# Autodesk Inventor assembly: Jose_Ensamble_Set_Sobre_Robot
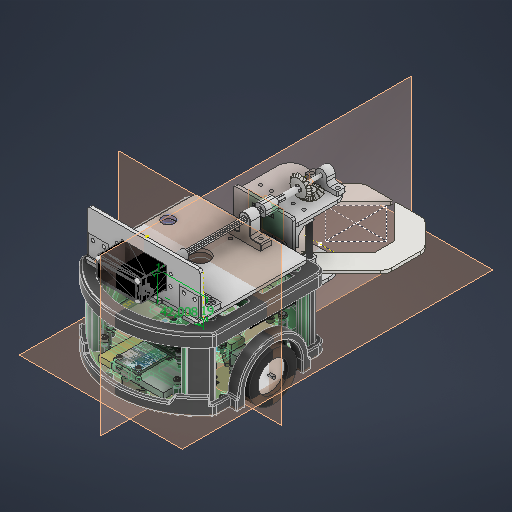
[picture p0: Inventor's stored thumbnail of the model, 512x512]
Saved by Autodesk Inventor 2026.3 (Build 303398000, 398)
## iProperties
Created: 2025-10-21
Part Number: Jose_Ensamble_Set_Sobre_Robot
Document SubType Name: Assembly
Designer: brene
Author: brene
## Documents named in this file (50)
- C:\Users\Caro\JoseCarlos\TEC\TFG\Inventor\PiezasSTD\Jose_Ensamble_Set_Sobre_Robot.iam
- C:\Users\Caro\JoseCarlos\TEC\TFG\Inventor\AttaBotStemV3\Diseño V3.0\base_chasis_v6\base_chasis_v4-dimsAjustadas.ipt
- C:\Users\Caro\JoseCarlos\TEC\TFG\Inventor\AttaBotStemV3\Diseño V3.0\base_chasis_v6.ipt
- C:\Users\Caro\JoseCarlos\TEC\TFG\Inventor\AttaBotStemV3\Diseño V3.0\Content Center Files\en-US\ISO 4762(2)\ISO 4762 - M2 x 12ISO.ipt
- C:\Users\Caro\JoseCarlos\TEC\TFG\Inventor\AttaBotStemV3\Diseño V3.0\switch.ipt
- C:\Users\Caro\JoseCarlos\TEC\TFG\Inventor\AttaBotStemV3\Diseño V3.0\Content Center Files\en-US\ISO 4762(2)\ISO 4762 - M2 x 8ISO.ipt
- C:\Users\Caro\JoseCarlos\TEC\TFG\Inventor\AttaBotStemV3\Diseño V3.0\Content Center Files\en-US\ISO 4032(2)\ISO 4032 - M2 - ISO.ipt
- C:\Users\Caro\JoseCarlos\TEC\TFG\Inventor\AttaBotStemV3\Diseño V3.0\ball_caster.ipt
- C:\Users\Caro\JoseCarlos\TEC\TFG\Inventor\AttaBotStemV3\Diseño V3.0\sensorInferior.ipt
- C:\Users\Caro\JoseCarlos\TEC\TFG\Inventor\AttaBotStemV3\Diseño V3.0\Content Center Files\en-US\ISO 4762(2)\ISO 4762 - M3 x 12ISO.ipt
- C:\Users\Caro\JoseCarlos\TEC\TFG\Inventor\AttaBotStemV3\Diseño V3.0\Content Center Files\en-US\ISO 4032(2)\ISO 4032 - M3 - ISO.ipt
- C:\Users\Caro\JoseCarlos\TEC\TFG\Inventor\AttaBotStemV3\Diseño V3.0\spacers\hexagonal_spacer_MF_M3_H20_HEX5.5_FTD6_MTL6.ipt
- C:\Users\Caro\JoseCarlos\TEC\TFG\Inventor\AttaBotStemV3\Diseño V3.0\spacers\hexagonal_spacer_MF_M3_H06_HEX5.5_FTD3_MTL6.ipt
- C:\Users\Caro\JoseCarlos\TEC\TFG\Inventor\AttaBotStemV3\Diseño V3.0\Content Center Files\en-US\ISO 4762(2)\ISO 4762 - M3 x 8ISO.ipt
- C:\Users\Caro\JoseCarlos\TEC\TFG\Inventor\AttaBotStemV3\Diseño V3.0\spacers\hexagonal_spacer_MF_M3_H08_HEX5_FTD4_MTL8.ipt
- C:\Users\Caro\JoseCarlos\TEC\TFG\Inventor\AttaBotStemV3\Diseño V3.0\bateria.ipt
- C:\Users\Caro\JoseCarlos\TEC\TFG\Inventor\AttaBotStemV3\Diseño V3.0\base_powerboost.ipt
- C:\Users\Caro\JoseCarlos\TEC\TFG\Inventor\AttaBotStemV3\Diseño V3.0\powerboost.ipt
- C:\Users\Caro\JoseCarlos\TEC\TFG\Inventor\AttaBotStemV3\Diseño V3.0\base_nivel2.ipt
- C:\Users\Caro\JoseCarlos\TEC\TFG\Inventor\AttaBotStemV3\Diseño V3.0\ideaboard.ipt
- C:\Users\Caro\JoseCarlos\TEC\TFG\Inventor\AttaBotStemV3\Diseño V3.0\sensorFrontal.ipt
- C:\Users\Caro\JoseCarlos\TEC\TFG\Inventor\AttaBotStemV3\Diseño V3.0\Tower Pro MG90S Micro servo.ipt
- C:\Users\Caro\JoseCarlos\TEC\TFG\Inventor\AttaBotStemV3\Diseño V3.0\spacers\hexagonal_spacer_MF_M3_H10_HEX5.5_FTD6_MTL6.ipt
- C:\Users\Caro\JoseCarlos\TEC\TFG\Inventor\AttaBotStemV3\Diseño V3.0\SoporteMotor_3.0.ipt
- C:\Users\Caro\JoseCarlos\TEC\TFG\Inventor\AttaBotStemV3\Diseño V3.0\motor.ipt
- C:\Users\Caro\JoseCarlos\TEC\TFG\Inventor\AttaBotStemV3\Diseño V3.0\llanta.ipt
- C:\Users\Caro\JoseCarlos\TEC\TFG\Inventor\AttaBotStemV3\Diseño V3.0\Unidirectional shoulder.ipt
- C:\Users\Caro\JoseCarlos\TEC\TFG\Inventor\AttaBotStemV3\Diseño V3.0\SujecionServo.ipt
- C:\Users\06aar\Documents\Inventor\Content Center Files\R2026\en-US\SS-ISO 4762\ISO 4762 - M2,5 x 25SS-ISO.ipt
- C:\Users\Caro\JoseCarlos\TEC\TFG\Inventor\AttaBotStemV3\Diseño V3.0\Esquinero Trasero\base_chasis_v4-dimsAjustadas.ipt
- C:\Users\Caro\JoseCarlos\TEC\TFG\Inventor\AttaBotStemV3\Diseño V3.0\Esquinero Trasero.ipt
- C:\Users\Caro\JoseCarlos\TEC\TFG\Inventor\AttaBotStemV3\Diseño V3.0\Bumper Trasero\base_chasis_v4-dimsAjustadas.ipt
- C:\Users\Caro\JoseCarlos\TEC\TFG\Inventor\AttaBotStemV3\Diseño V3.0\Bumper Trasero.ipt
- C:\Users\Caro\JoseCarlos\TEC\TFG\Inventor\AttaBotStemV3\Diseño V3.0\Guardabarros.ipt
- C:\Users\Caro\JoseCarlos\TEC\TFG\Inventor\AttaBotStemV3\Diseño V3.0\Bumper Delantero.ipt
- C:\Users\Caro\JoseCarlos\TEC\TFG\Inventor\AttaBotStemV3\Diseño V3.0\Esquineros Delanteros.ipt
- C:\Users\Caro\JoseCarlos\TEC\TFG\Inventor\AttaBotStemV3\Diseño V3.0\PARED TRASERA.ipt
- C:\Users\Caro\JoseCarlos\TEC\TFG\Inventor\AttaBotStemV3\Diseño V3.0\PAREDES LATERALES.ipt
- C:\Users\Caro\JoseCarlos\TEC\TFG\Inventor\AttaBotStemV3\Diseño V3.0\PAREDES LATERALES_MIR.ipt
- C:\Users\Caro\JoseCarlos\TEC\TFG\Inventor\AttaBotStemV3\Diseño V3.0\PARED FRONTAL.ipt
- C:\Users\Caro\JoseCarlos\TEC\TFG\Inventor\AttaBotStemV3\Diseño V3.0\Techo Armadura.ipt
- C:\Users\Caro\JoseCarlos\TEC\TFG\Inventor\AttaBotStemV3\Diseño V3.0\Acrilicos Superiores.ipt
- C:\Users\Caro\JoseCarlos\TEC\TFG\Inventor\AttaBotStemV3\Diseño V3.0\Pieza de Silicona.ipt
- C:\Users\Caro\JoseCarlos\TEC\TFG\Inventor\AttaBotStemV3\Diseño V3.0\PresaPilotInventorVersion.ipt
- C:\Users\Caro\JoseCarlos\TEC\TFG\Inventor\AttaBotStemV3\Diseño V3.0\spacers\hexagonal_spacer_MF_M3_H20_HEX5.5_FTD6_MTL6_MIR.ipt
- C:\Users\Caro\JoseCarlos\TEC\TFG\Inventor\PiezasSTD\BaseMotorSetJose.ipt
- C:\Users\Caro\JoseCarlos\TEC\TFG\Inventor\PiezasSTD\EnsambleGarraSTD.iam
- C:\Users\Caro\JoseCarlos\TEC\TFG\Inventor\PiezasSTD\DistanciaSpacer3mm.ipt
- C:\Users\Caro\JoseCarlos\TEC\TFG\Inventor\PiezasSTD\EnsambleMotor\EnsambleBaseMotor.iam
- C:\Users\Caro\JoseCarlos\TEC\TFG\Inventor\PiezasSTD\EnsambleMotor\EjeMotor.ipt
## Components (120 placed, 44 different names)
1. BaseMotorSetJose:1 — Nivelación:215
2. EnsambleGarraSTD:1 [sub-assembly] — Coincidencia:293, Nivelación:220, Coincidencia:294, Nivelación:222
3. DistanciaSpacer3mm:1 — Nivelación:219, Coincidencia:293
4. EjeMotor:1 — Nivelación:222
5. EnsambleBaseMotor_Mediciones [sub-assembly] — Ángulo:7, Coincidencia:299, Coincidencia:300, Ángulo:8
6. hexagonal_spacer_MF_M3_H20_HEX5.5_FTD6_MTL6:5 — Coincidencia:289, Coincidencia:290
7. hexagonal_spacer_MF_M3_H20_HEX5.5_FTD6_MTL6_MIR:1
8. ISO 4762 M3 x 8:10 — Coincidencia:151, Coincidencia:152
9. ISO 4762 M3 x 8:9 — Coincidencia:153, Coincidencia:154, Coincidencia:285
10. hexagonal_spacer_MF_M3_H10_HEX5.5_FTD6_MTL6:2 — Coincidencia:148, Coincidencia:150
11. hexagonal_spacer_MF_M3_H10_HEX5.5_FTD6_MTL6:1 — Coincidencia:147, Coincidencia:149
12. ISO 4762 M3 x 8:8 — Coincidencia:113, Coincidencia:114, Coincidencia:250, Coincidencia:251
13. ISO 4762 M3 x 8:7 — Coincidencia:117, Coincidencia:118
14. ISO 4032 M3:8 — Coincidencia:123, Coincidencia:124
15. ISO 4032 M3:7 — Coincidencia:125, Coincidencia:126
16. hexagonal_spacer_MF_M3_H06_HEX5.5_FTD3_MTL6:10 — Coincidencia:115, Coincidencia:116, Coincidencia:119, Coincidencia:120, Coincidencia:126
17. hexagonal_spacer_MF_M3_H06_HEX5.5_FTD3_MTL6:9 — Coincidencia:111, Coincidencia:112, Coincidencia:121, Coincidencia:122, Coincidencia:124
18. hexagonal_spacer_MF_M3_H06_HEX5.5_FTD3_MTL6:8 — Coincidencia:104, Coincidencia:105, Coincidencia:108, Coincidencia:110, Coincidencia:132, Coincidencia:175
19. hexagonal_spacer_MF_M3_H06_HEX5.5_FTD3_MTL6:7 — Coincidencia:106, Coincidencia:107, Coincidencia:134, Coincidencia:177
20. hexagonal_spacer_MF_M3_H06_HEX5.5_FTD3_MTL6:6 — Coincidencia:100, Coincidencia:101, Coincidencia:109, Coincidencia:130, Coincidencia:179, Coincidencia:275, Coincidencia:276, Coincidencia:277, Coincidencia:278, Coincidencia:279, Coincidencia:280, Coincidencia:281
21. hexagonal_spacer_MF_M3_H06_HEX5.5_FTD3_MTL6:5 — Coincidencia:102, Coincidencia:103, Coincidencia:128, Coincidencia:181
22. ISO 4762 M3 x 8:6 — Coincidencia:94, Coincidencia:95
23. ISO 4762 M3 x 8:5 — Coincidencia:96, Coincidencia:97
24. ISO 4762 M3 x 8:4 — Coincidencia:92, Coincidencia:93
25. ISO 4762 M3 x 8:3 — Coincidencia:98, Coincidencia:99
26. ISO 4032 M2:10 — Coincidencia:84, Coincidencia:85
27. ISO 4032 M2:9 — Coincidencia:80, Coincidencia:81
28. ISO 4032 M2:8 — Coincidencia:86, Coincidencia:87
29. ISO 4032 M2:7 — Coincidencia:82, Coincidencia:83
30. ISO 4032 M2:6 — Coincidencia:64, Coincidencia:65, Coincidencia:70
31. ISO 4032 M2:5 — Coincidencia:66, Coincidencia:67
32. ISO 4032 M2:4 — Coincidencia:62, Coincidencia:63, Coincidencia:71
33. ISO 4032 M2:3 — Coincidencia:68, Coincidencia:69
34. ISO 4762 M2 x 8:6 — Coincidencia:76, Coincidencia:77, Coincidencia:87, Coincidencia:91
35. ISO 4762 M2 x 8:5 — Coincidencia:78, Coincidencia:79, Coincidencia:85
36. ISO 4762 M2 x 12:2 — Coincidencia:72, Coincidencia:73, Coincidencia:83
37. ISO 4762 M2 x 12:1 — Coincidencia:74, Coincidencia:75, Coincidencia:81
38. ISO 4032 M3:6 — Coincidencia:48, Coincidencia:49, Coincidencia:57
39. ISO 4032 M3:5 — Coincidencia:50, Coincidencia:51, Coincidencia:59
40. ISO 4032 M3:4 — Coincidencia:46, Coincidencia:47, Coincidencia:53
41. ISO 4032 M3:3 — Coincidencia:44, Coincidencia:45, Coincidencia:55
42. hexagonal_spacer_MF_M3_H08_HEX5_FTD4_MTL8:4 — Coincidencia:54, Coincidencia:55, Coincidencia:90
43. hexagonal_spacer_MF_M3_H08_HEX5_FTD4_MTL8:3 — Coincidencia:52, Coincidencia:53, Coincidencia:89
44. hexagonal_spacer_MF_M3_H08_HEX5_FTD4_MTL8:2 — Coincidencia:58, Coincidencia:59, Coincidencia:88
45. hexagonal_spacer_MF_M3_H08_HEX5_FTD4_MTL8:1 — Coincidencia:56, Coincidencia:57, Coincidencia:61
46. ISO 4762 M3 x 8:2 — Coincidencia:34, Coincidencia:35, Coincidencia:39
47. ISO 4762 M3 x 8:1 — Coincidencia:32, Coincidencia:33, Coincidencia:37
48. hexagonal_spacer_MF_M3_H20_HEX5.5_FTD6_MTL6:4 — Coincidencia:36, Coincidencia:37, Coincidencia:137, Coincidencia:145
49. hexagonal_spacer_MF_M3_H20_HEX5.5_FTD6_MTL6:3 — Coincidencia:38, Coincidencia:39, Coincidencia:143
50. hexagonal_spacer_MF_M3_H20_HEX5.5_FTD6_MTL6:2 — Coincidencia:26, Coincidencia:27, Coincidencia:135, Coincidencia:141
51. hexagonal_spacer_MF_M3_H20_HEX5.5_FTD6_MTL6:1 — Coincidencia:24, Coincidencia:25, Coincidencia:136, Coincidencia:139
52. ISO 4032 M3:2 — Coincidencia:14, Coincidencia:15, Coincidencia:23
53. ISO 4032 M3:1 — Coincidencia:12, Coincidencia:13, Coincidencia:21
54. ISO 4762 M3 x 12:2 — Coincidencia:23, Coincidencia:27
55. ISO 4762 M3 x 12:1 — Coincidencia:21, Coincidencia:25, Coincidencia:283
56. ISO 4762 M2 x 8:4 — Coincidencia:8, Coincidencia:9, Tangente:4
57. ISO 4762 M2 x 8:3 — Coincidencia:10, Coincidencia:11, Tangente:3
58. ISO 4032 M2:2 — Insertar:2
59. ISO 4032 M2:1 — Insertar:1
60. ISO 4762 M2 x 8:2 — Coincidencia:3, Coincidencia:4
61. ISO 4762 M2 x 8:1 — Coincidencia:5, Coincidencia:6
62. ISO 4032 M3:16 — Coincidencia:144, Coincidencia:145
63. ISO 4032 M3:15 — Coincidencia:140, Coincidencia:141
64. ISO 4032 M3:14 — Coincidencia:138, Coincidencia:139
65. ISO 4032 M3:13 — Coincidencia:142, Coincidencia:143
66. ISO 4032 M3:12 — Coincidencia:127, Coincidencia:128
67. ISO 4032 M3:11 — Coincidencia:131, Coincidencia:132
68. ISO 4032 M3:10 — Coincidencia:129, Coincidencia:130
69. ISO 4032 M3:9 — Coincidencia:133, Coincidencia:134
70. ISO 4032 M2:15 — Coincidencia:194, Coincidencia:195
71. ISO 4032 M2:14 — Coincidencia:196, Coincidencia:197
72. ISO 4032 M2:13 — Coincidencia:192, Coincidencia:193
73. ISO 4032 M2:12 — Coincidencia:190, Coincidencia:191
74. ISO 4762 M2 x 8:10 — Coincidencia:183, Coincidencia:197
75. ISO 4762 M2 x 8:9 — Coincidencia:187, Coincidencia:193
76. ISO 4762 M2 x 8:8 — Coincidencia:189, Coincidencia:191
77. ISO 4762 M2 x 8:7 — Coincidencia:185, Coincidencia:195
78. ISO 4762 M3 x 8:14 — Coincidencia:174, Coincidencia:175
79. ISO 4762 M3 x 8:13 — Coincidencia:178, Coincidencia:179
80. ISO 4762 M3 x 8:12 — Coincidencia:180, Coincidencia:181, Coincidencia:274
81. ISO 4762 M3 x 8:11 — Coincidencia:176, Coincidencia:177
82. SS ISO 4762 M2,5 x 25:12 — Insert:18, Coincidencia:282
83. SS ISO 4762 M2,5 x 25:11 — Insert:17
84. SS ISO 4762 M2,5 x 25:9 — Insert:15
85. SS ISO 4762 M2,5 x 25:8 — Insert:14
86. SS ISO 4762 M2,5 x 25:6 — Insert:12
87. SS ISO 4762 M2,5 x 25:4 — Insert:10
88. sensorInferior:3 — Coincidencia:282, Coincidencia:283, Coincidencia:284
89. switch:1 — Coincidencia:1, Coincidencia:2, Coincidencia:3, Coincidencia:5, Ángulo:3
90. ball_caster:1 — Coincidencia:7, Tangente:1, Tangente:2, Coincidencia:9, Coincidencia:11
91. bateria:1 — Coincidencia:60, Coincidencia:61, Coincidencia:146, Ángulo:2
92. base_powerboost:1 — Coincidencia:62, Coincidencia:63, Coincidencia:64, Coincidencia:65, Coincidencia:66, Coincidencia:67, Coincidencia:68, Coincidencia:69, Coincidencia:80, Coincidencia:82, Coincidencia:84, Coincidencia:86, Coincidencia:88, Coincidencia:89, Coincidencia:90, Coincidencia:91, Coincidencia:92, Coincidencia:93, Coincidencia:94, Coincidencia:95, Coincidencia:96, Coincidencia:97, Coincidencia:98, Coincidencia:99
93. powerboost:1 — Coincidencia:70, Coincidencia:71, Coincidencia:72, Coincidencia:73, Coincidencia:74, Coincidencia:75, Coincidencia:76, Coincidencia:77, Coincidencia:78, Coincidencia:79
94. base_nivel2:1 — Coincidencia:100, Coincidencia:101, Coincidencia:102, Coincidencia:103, Coincidencia:104, Coincidencia:105, Coincidencia:106, Coincidencia:107, Coincidencia:111, Coincidencia:112, Coincidencia:113, Coincidencia:114, Coincidencia:115, Coincidencia:116, Coincidencia:117, Coincidencia:118, Coincidencia:127, Coincidencia:129, Coincidencia:131, Coincidencia:133, Coincidencia:135, Coincidencia:136, Coincidencia:137, Coincidencia:138, Coincidencia:140, Coincidencia:142, Coincidencia:144, Ángulo:4, Ángulo:5, Coincidencia:250, Coincidencia:251, Coincidencia:274, Coincidencia:275, Coincidencia:276, Coincidencia:277, Coincidencia:278, Coincidencia:279, Coincidencia:280, Coincidencia:281
95. ideaboard:1 — Coincidencia:108, Coincidencia:109, Coincidencia:110, Coincidencia:174, Coincidencia:176, Coincidencia:178, Coincidencia:180
96. sensorFrontal:1 — Coincidencia:121, Coincidencia:122, Coincidencia:123, Ángulo:5
97. motor:1 — Coincidencia:161, Coincidencia:163, Coincidencia:164, Coincidencia:227, Tangente:5
98. sensorFrontal:2 — Coincidencia:119, Coincidencia:120, Coincidencia:125, Ángulo:4
99. motor:2 — Coincidencia:169, Coincidencia:171, Coincidencia:172, Coincidencia:230, Tangente:6
100. llanta:1 — Coincidencia:163, Coincidencia:164, Coincidencia:272
101. llanta:2 — Coincidencia:171, Coincidencia:172
102. Tower Pro MG90S Micro servo:2 — Coincidencia:205, Coincidencia:206, Coincidencia:207, Ángulo:1, Coincidencia:217
103. Unidirectional shoulder:1 — Coincidencia:205, Coincidencia:206
104. SujecionServo:1 — Coincidencia:217
105. SoporteMotor_3.0:1 — Coincidencia:229, Coincidencia:230, Coincidencia:231, Coincidencia:233, Tangente:6
106. SoporteMotor_3.0:2 — Coincidencia:226, Coincidencia:227, Coincidencia:228, Tangente:5, Coincidencia:232
107. PARED TRASERA:1 — Coincidencia:253, Coincidencia:254
108. PAREDES LATERALES:2 — Coincidencia:255, Coincidencia:256, Coincidencia:257
109. PAREDES LATERALES_MIR:1
110. PARED FRONTAL:1 — Coincidencia:258, Coincidencia:259, Coincidencia:260, Coincidencia:269, Nivelación:219
111. Acrilicos Superiores:1 — Coincidencia:291, Coincidencia:292, Nivelación:216, Coincidencia:295, Coincidencia:296, Coincidencia:297, Coincidencia:298, Coincidencia:299
112. base_chasis_v4-dimsAjustadas:3 — Nivelación:212, Coincidencia:237, Coincidencia:238, Coincidencia:256, Coincidencia:261, Coincidencia:263, Coincidencia:264
113. base_chasis_v4-dimsAjustadas:1 — Coincidencia:239, Coincidencia:240, Coincidencia:244, Coincidencia:254
114. base_chasis_v4-dimsAjustadas:2 — Coincidencia:1, Coincidencia:2, Coincidencia:4, Coincidencia:6, Insertar:1, Insertar:2, Coincidencia:7, Tangente:1, Tangente:2, Coincidencia:8, Coincidencia:10, Tangente:3, Tangente:4, Coincidencia:12, Coincidencia:13, Coincidencia:14, Coincidencia:15, Coincidencia:24, Coincidencia:26, Coincidencia:32, Coincidencia:33, Coincidencia:34, Coincidencia:35, Coincidencia:36, Coincidencia:38, Coincidencia:44, Coincidencia:45, Coincidencia:46, Coincidencia:47, Coincidencia:48, Coincidencia:49, Coincidencia:50, Coincidencia:51, Coincidencia:52, Coincidencia:54, Coincidencia:56, Coincidencia:58, Coincidencia:60, Coincidencia:146, Coincidencia:147, Coincidencia:148, Coincidencia:149, Coincidencia:150, Coincidencia:151, Coincidencia:152, Coincidencia:153, Coincidencia:154, Coincidencia:161, Coincidencia:169, Coincidencia:183, Coincidencia:185, Coincidencia:187, Coincidencia:189, Coincidencia:190, Coincidencia:192, Coincidencia:194, Coincidencia:196, Coincidencia:207, Ángulo:1, Coincidencia:209, Nivelación:211, Coincidencia:210, Ángulo:2, Ángulo:3, Coincidencia:226, Coincidencia:228, Coincidencia:229, Coincidencia:231, Coincidencia:232, Coincidencia:233, Insert:10, Insert:12, Insert:14, Insert:15, Insert:17, Insert:18, Nivelación:212, Coincidencia:237, Coincidencia:238, Coincidencia:239, Coincidencia:240, Coincidencia:244, Coincidencia:245, Coincidencia:246, Coincidencia:247, Coincidencia:249, Coincidencia:253, Coincidencia:255, Coincidencia:258, Coincidencia:262, Coincidencia:270, Coincidencia:273, Coincidencia:284, Coincidencia:285, Coincidencia:286, Coincidencia:287, Coincidencia:289, Coincidencia:290, Coincidencia:300
115. Guardabarros:1 — Coincidencia:270, Coincidencia:272, Coincidencia:273
116. Pieza de Silicona:1 — Nivelación:213, Coincidencia:268
117. PresaPilotInventorVersion:1 — Coincidencia:286, Coincidencia:287, Coincidencia:288
118. Bumper Delantero:1 — Coincidencia:245, Coincidencia:246, Coincidencia:247, Coincidencia:248, Coincidencia:252, Coincidencia:259, Nivelación:220
119. Esquineros Delanteros:1 — Coincidencia:248, Coincidencia:249, Coincidencia:252, Coincidencia:257, Coincidencia:260, Coincidencia:269, Coincidencia:291
120. Techo Armadura:1 — Coincidencia:261, Coincidencia:262, Coincidencia:263, Coincidencia:264, Nivelación:213, Coincidencia:268, Coincidencia:292, Coincidencia:295, Coincidencia:296, Coincidencia:297, Coincidencia:298, Ángulo:6
## Relationships (267: Mate 237, Insert 8, Angle 8, Flush 8, Tangent 6)
- Coincidencia:1 [Mate]: switch:1 ↔ base_chasis_v4-dimsAjustadas:2
- Coincidencia:2 [Mate]: switch:1 ↔ base_chasis_v4-dimsAjustadas:2
- Coincidencia:3 [Mate]: ISO 4762 M2 x 8:2 ↔ switch:1
- Coincidencia:4 [Mate]: ISO 4762 M2 x 8:2 ↔ base_chasis_v4-dimsAjustadas:2
- Coincidencia:5 [Mate]: ISO 4762 M2 x 8:1 ↔ switch:1
- Coincidencia:6 [Mate]: ISO 4762 M2 x 8:1 ↔ base_chasis_v4-dimsAjustadas:2
- Insertar:1: ISO 4032 M2:1 ↔ base_chasis_v4-dimsAjustadas:2
- Insertar:2: ISO 4032 M2:2 ↔ base_chasis_v4-dimsAjustadas:2
- Coincidencia:7 [Mate]: ball_caster:1 ↔ base_chasis_v4-dimsAjustadas:2
- Tangente:1: ball_caster:1 ↔ base_chasis_v4-dimsAjustadas:2
- Tangente:2: ball_caster:1 ↔ base_chasis_v4-dimsAjustadas:2
- Coincidencia:8 [Mate]: ISO 4762 M2 x 8:4 ↔ base_chasis_v4-dimsAjustadas:2
- Coincidencia:9 [Mate]: ISO 4762 M2 x 8:4 ↔ ball_caster:1
- Coincidencia:10 [Mate]: ISO 4762 M2 x 8:3 ↔ base_chasis_v4-dimsAjustadas:2
- Coincidencia:11 [Mate]: ISO 4762 M2 x 8:3 ↔ ball_caster:1
- Tangente:3: ISO 4762 M2 x 8:3 ↔ base_chasis_v4-dimsAjustadas:2
- Tangente:4: ISO 4762 M2 x 8:4 ↔ base_chasis_v4-dimsAjustadas:2
- Coincidencia:12 [Mate]: ISO 4032 M3:1 ↔ base_chasis_v4-dimsAjustadas:2
- Coincidencia:13 [Mate]: ISO 4032 M3:1 ↔ base_chasis_v4-dimsAjustadas:2
- Coincidencia:14 [Mate]: ISO 4032 M3:2 ↔ base_chasis_v4-dimsAjustadas:2
- Coincidencia:15 [Mate]: ISO 4032 M3:2 ↔ base_chasis_v4-dimsAjustadas:2
- Coincidencia:21 [Mate]: ISO 4032 M3:1 ↔ ISO 4762 M3 x 12:1
- Coincidencia:23 [Mate]: ISO 4032 M3:2 ↔ ISO 4762 M3 x 12:2
- Coincidencia:24 [Mate]: hexagonal_spacer_MF_M3_H20_HEX5.5_FTD6_MTL6:1 ↔ base_chasis_v4-dimsAjustadas:2
- Coincidencia:25 [Mate]: hexagonal_spacer_MF_M3_H20_HEX5.5_FTD6_MTL6:1 ↔ ISO 4762 M3 x 12:1
- Coincidencia:26 [Mate]: hexagonal_spacer_MF_M3_H20_HEX5.5_FTD6_MTL6:2 ↔ base_chasis_v4-dimsAjustadas:2
- Coincidencia:27 [Mate]: hexagonal_spacer_MF_M3_H20_HEX5.5_FTD6_MTL6:2 ↔ ISO 4762 M3 x 12:2
- Coincidencia:32 [Mate]: ISO 4762 M3 x 8:1 ↔ base_chasis_v4-dimsAjustadas:2
- Coincidencia:33 [Mate]: ISO 4762 M3 x 8:1 ↔ base_chasis_v4-dimsAjustadas:2
- Coincidencia:34 [Mate]: ISO 4762 M3 x 8:2 ↔ base_chasis_v4-dimsAjustadas:2
- Coincidencia:35 [Mate]: ISO 4762 M3 x 8:2 ↔ base_chasis_v4-dimsAjustadas:2
- Coincidencia:36 [Mate]: hexagonal_spacer_MF_M3_H20_HEX5.5_FTD6_MTL6:4 ↔ base_chasis_v4-dimsAjustadas:2
- Coincidencia:37 [Mate]: ISO 4762 M3 x 8:1 ↔ hexagonal_spacer_MF_M3_H20_HEX5.5_FTD6_MTL6:4
- Coincidencia:38 [Mate]: hexagonal_spacer_MF_M3_H20_HEX5.5_FTD6_MTL6:3 ↔ base_chasis_v4-dimsAjustadas:2
- Coincidencia:39 [Mate]: ISO 4762 M3 x 8:2 ↔ hexagonal_spacer_MF_M3_H20_HEX5.5_FTD6_MTL6:3
- Coincidencia:44 [Mate]: ISO 4032 M3:3 ↔ base_chasis_v4-dimsAjustadas:2
- Coincidencia:45 [Mate]: ISO 4032 M3:3 ↔ base_chasis_v4-dimsAjustadas:2
- Coincidencia:46 [Mate]: ISO 4032 M3:4 ↔ base_chasis_v4-dimsAjustadas:2
- Coincidencia:47 [Mate]: ISO 4032 M3:4 ↔ base_chasis_v4-dimsAjustadas:2
- Coincidencia:48 [Mate]: ISO 4032 M3:6 ↔ base_chasis_v4-dimsAjustadas:2
- Coincidencia:49 [Mate]: ISO 4032 M3:6 ↔ base_chasis_v4-dimsAjustadas:2
- Coincidencia:50 [Mate]: ISO 4032 M3:5 ↔ base_chasis_v4-dimsAjustadas:2
- Coincidencia:51 [Mate]: ISO 4032 M3:5 ↔ base_chasis_v4-dimsAjustadas:2
- Coincidencia:52 [Mate]: hexagonal_spacer_MF_M3_H08_HEX5_FTD4_MTL8:3 ↔ base_chasis_v4-dimsAjustadas:2
- Coincidencia:53 [Mate]: ISO 4032 M3:4 ↔ hexagonal_spacer_MF_M3_H08_HEX5_FTD4_MTL8:3
- Coincidencia:54 [Mate]: hexagonal_spacer_MF_M3_H08_HEX5_FTD4_MTL8:4 ↔ base_chasis_v4-dimsAjustadas:2
- Coincidencia:55 [Mate]: ISO 4032 M3:3 ↔ hexagonal_spacer_MF_M3_H08_HEX5_FTD4_MTL8:4
- Coincidencia:56 [Mate]: hexagonal_spacer_MF_M3_H08_HEX5_FTD4_MTL8:1 ↔ base_chasis_v4-dimsAjustadas:2
- Coincidencia:57 [Mate]: ISO 4032 M3:6 ↔ hexagonal_spacer_MF_M3_H08_HEX5_FTD4_MTL8:1
- Coincidencia:58 [Mate]: hexagonal_spacer_MF_M3_H08_HEX5_FTD4_MTL8:2 ↔ base_chasis_v4-dimsAjustadas:2
- Coincidencia:59 [Mate]: ISO 4032 M3:5 ↔ hexagonal_spacer_MF_M3_H08_HEX5_FTD4_MTL8:2
- Coincidencia:60 [Mate]: bateria:1 ↔ base_chasis_v4-dimsAjustadas:2
- Coincidencia:61 [Mate]: hexagonal_spacer_MF_M3_H08_HEX5_FTD4_MTL8:1 ↔ bateria:1
- Coincidencia:62 [Mate]: ISO 4032 M2:4 ↔ base_powerboost:1
- Coincidencia:63 [Mate]: ISO 4032 M2:4 ↔ base_powerboost:1
- Coincidencia:64 [Mate]: ISO 4032 M2:6 ↔ base_powerboost:1
- Coincidencia:65 [Mate]: ISO 4032 M2:6 ↔ base_powerboost:1
- Coincidencia:66 [Mate]: ISO 4032 M2:5 ↔ base_powerboost:1
- Coincidencia:67 [Mate]: ISO 4032 M2:5 ↔ base_powerboost:1
- Coincidencia:68 [Mate]: ISO 4032 M2:3 ↔ base_powerboost:1
- Coincidencia:69 [Mate]: ISO 4032 M2:3 ↔ base_powerboost:1
- Coincidencia:70 [Mate]: ISO 4032 M2:6 ↔ powerboost:1
- Coincidencia:71 [Mate]: ISO 4032 M2:4 ↔ powerboost:1
- Coincidencia:72 [Mate]: ISO 4762 M2 x 12:2 ↔ powerboost:1
- Coincidencia:73 [Mate]: ISO 4762 M2 x 12:2 ↔ powerboost:1
- Coincidencia:74 [Mate]: ISO 4762 M2 x 12:1 ↔ powerboost:1
- Coincidencia:75 [Mate]: ISO 4762 M2 x 12:1 ↔ powerboost:1
- Coincidencia:76 [Mate]: ISO 4762 M2 x 8:6 ↔ powerboost:1
- Coincidencia:77 [Mate]: ISO 4762 M2 x 8:6 ↔ powerboost:1
- Coincidencia:78 [Mate]: ISO 4762 M2 x 8:5 ↔ powerboost:1
- Coincidencia:79 [Mate]: ISO 4762 M2 x 8:5 ↔ powerboost:1
- Coincidencia:80 [Mate]: ISO 4032 M2:9 ↔ base_powerboost:1
- Coincidencia:81 [Mate]: ISO 4032 M2:9 ↔ ISO 4762 M2 x 12:1
- Coincidencia:82 [Mate]: ISO 4032 M2:7 ↔ base_powerboost:1
- Coincidencia:83 [Mate]: ISO 4032 M2:7 ↔ ISO 4762 M2 x 12:2
- Coincidencia:84 [Mate]: ISO 4032 M2:10 ↔ base_powerboost:1
- Coincidencia:85 [Mate]: ISO 4032 M2:10 ↔ ISO 4762 M2 x 8:5
- Coincidencia:86 [Mate]: ISO 4032 M2:8 ↔ base_powerboost:1
- Coincidencia:87 [Mate]: ISO 4032 M2:8 ↔ ISO 4762 M2 x 8:6
- Coincidencia:88 [Mate]: hexagonal_spacer_MF_M3_H08_HEX5_FTD4_MTL8:2 ↔ base_powerboost:1
- Coincidencia:89 [Mate]: hexagonal_spacer_MF_M3_H08_HEX5_FTD4_MTL8:3 ↔ base_powerboost:1
- Coincidencia:90 [Mate]: hexagonal_spacer_MF_M3_H08_HEX5_FTD4_MTL8:4 ↔ base_powerboost:1
- Coincidencia:91 [Mate]: ISO 4762 M2 x 8:6 ↔ base_powerboost:1
- Coincidencia:92 [Mate]: ISO 4762 M3 x 8:4 ↔ base_powerboost:1
- Coincidencia:93 [Mate]: ISO 4762 M3 x 8:4 ↔ base_powerboost:1
- Coincidencia:94 [Mate]: ISO 4762 M3 x 8:6 ↔ base_powerboost:1
- Coincidencia:95 [Mate]: ISO 4762 M3 x 8:6 ↔ base_powerboost:1
- Coincidencia:96 [Mate]: ISO 4762 M3 x 8:5 ↔ base_powerboost:1
- Coincidencia:97 [Mate]: ISO 4762 M3 x 8:5 ↔ base_powerboost:1
- Coincidencia:98 [Mate]: ISO 4762 M3 x 8:3 ↔ base_powerboost:1
- Coincidencia:99 [Mate]: ISO 4762 M3 x 8:3 ↔ base_powerboost:1
- Coincidencia:100 [Mate]: hexagonal_spacer_MF_M3_H06_HEX5.5_FTD3_MTL6:6 ↔ base_nivel2:1
- Coincidencia:101 [Mate]: hexagonal_spacer_MF_M3_H06_HEX5.5_FTD3_MTL6:6 ↔ base_nivel2:1
- Coincidencia:102 [Mate]: hexagonal_spacer_MF_M3_H06_HEX5.5_FTD3_MTL6:5 ↔ base_nivel2:1
- Coincidencia:103 [Mate]: hexagonal_spacer_MF_M3_H06_HEX5.5_FTD3_MTL6:5 ↔ base_nivel2:1
- Coincidencia:104 [Mate]: hexagonal_spacer_MF_M3_H06_HEX5.5_FTD3_MTL6:8 ↔ base_nivel2:1
- Coincidencia:105 [Mate]: hexagonal_spacer_MF_M3_H06_HEX5.5_FTD3_MTL6:8 ↔ base_nivel2:1
- Coincidencia:106 [Mate]: hexagonal_spacer_MF_M3_H06_HEX5.5_FTD3_MTL6:7 ↔ base_nivel2:1
- Coincidencia:107 [Mate]: hexagonal_spacer_MF_M3_H06_HEX5.5_FTD3_MTL6:7 ↔ base_nivel2:1
- Coincidencia:108 [Mate]: hexagonal_spacer_MF_M3_H06_HEX5.5_FTD3_MTL6:8 ↔ ideaboard:1
- Coincidencia:109 [Mate]: hexagonal_spacer_MF_M3_H06_HEX5.5_FTD3_MTL6:6 ↔ ideaboard:1
- Coincidencia:110 [Mate]: hexagonal_spacer_MF_M3_H06_HEX5.5_FTD3_MTL6:8 ↔ ideaboard:1
- Coincidencia:111 [Mate]: hexagonal_spacer_MF_M3_H06_HEX5.5_FTD3_MTL6:9 ↔ base_nivel2:1
- Coincidencia:112 [Mate]: hexagonal_spacer_MF_M3_H06_HEX5.5_FTD3_MTL6:9 ↔ base_nivel2:1
- Coincidencia:113 [Mate]: ISO 4762 M3 x 8:8 ↔ base_nivel2:1
- Coincidencia:114 [Mate]: ISO 4762 M3 x 8:8 ↔ base_nivel2:1
- Coincidencia:115 [Mate]: hexagonal_spacer_MF_M3_H06_HEX5.5_FTD3_MTL6:10 ↔ base_nivel2:1
- Coincidencia:116 [Mate]: hexagonal_spacer_MF_M3_H06_HEX5.5_FTD3_MTL6:10 ↔ base_nivel2:1
- Coincidencia:117 [Mate]: ISO 4762 M3 x 8:7 ↔ base_nivel2:1
- Coincidencia:118 [Mate]: ISO 4762 M3 x 8:7 ↔ base_nivel2:1
- Coincidencia:119 [Mate]: hexagonal_spacer_MF_M3_H06_HEX5.5_FTD3_MTL6:10 ↔ sensorFrontal:2
- Coincidencia:120 [Mate]: hexagonal_spacer_MF_M3_H06_HEX5.5_FTD3_MTL6:10 ↔ sensorFrontal:2
- Coincidencia:121 [Mate]: hexagonal_spacer_MF_M3_H06_HEX5.5_FTD3_MTL6:9 ↔ sensorFrontal:1
- Coincidencia:122 [Mate]: hexagonal_spacer_MF_M3_H06_HEX5.5_FTD3_MTL6:9 ↔ sensorFrontal:1
- Coincidencia:123 [Mate]: ISO 4032 M3:8 ↔ sensorFrontal:1
- Coincidencia:124 [Mate]: ISO 4032 M3:8 ↔ hexagonal_spacer_MF_M3_H06_HEX5.5_FTD3_MTL6:9
- Coincidencia:125 [Mate]: ISO 4032 M3:7 ↔ sensorFrontal:2
- Coincidencia:126 [Mate]: ISO 4032 M3:7 ↔ hexagonal_spacer_MF_M3_H06_HEX5.5_FTD3_MTL6:10
- Coincidencia:127 [Mate]: ISO 4032 M3:12 ↔ base_nivel2:1
- Coincidencia:128 [Mate]: hexagonal_spacer_MF_M3_H06_HEX5.5_FTD3_MTL6:5 ↔ ISO 4032 M3:12
- Coincidencia:129 [Mate]: ISO 4032 M3:10 ↔ base_nivel2:1
- Coincidencia:130 [Mate]: hexagonal_spacer_MF_M3_H06_HEX5.5_FTD3_MTL6:6 ↔ ISO 4032 M3:10
- Coincidencia:131 [Mate]: ISO 4032 M3:11 ↔ base_nivel2:1
- Coincidencia:132 [Mate]: hexagonal_spacer_MF_M3_H06_HEX5.5_FTD3_MTL6:8 ↔ ISO 4032 M3:11
- Coincidencia:133 [Mate]: ISO 4032 M3:9 ↔ base_nivel2:1
- Coincidencia:134 [Mate]: hexagonal_spacer_MF_M3_H06_HEX5.5_FTD3_MTL6:7 ↔ ISO 4032 M3:9
- Coincidencia:135 [Mate]: hexagonal_spacer_MF_M3_H20_HEX5.5_FTD6_MTL6:2 ↔ base_nivel2:1
- Coincidencia:136 [Mate]: hexagonal_spacer_MF_M3_H20_HEX5.5_FTD6_MTL6:1 ↔ base_nivel2:1
- Coincidencia:137 [Mate]: hexagonal_spacer_MF_M3_H20_HEX5.5_FTD6_MTL6:4 ↔ base_nivel2:1
- Coincidencia:138 [Mate]: ISO 4032 M3:14 ↔ base_nivel2:1
- Coincidencia:139 [Mate]: hexagonal_spacer_MF_M3_H20_HEX5.5_FTD6_MTL6:1 ↔ ISO 4032 M3:14
- Coincidencia:140 [Mate]: ISO 4032 M3:15 ↔ base_nivel2:1
- Coincidencia:141 [Mate]: hexagonal_spacer_MF_M3_H20_HEX5.5_FTD6_MTL6:2 ↔ ISO 4032 M3:15
- Coincidencia:142 [Mate]: ISO 4032 M3:13 ↔ base_nivel2:1
- Coincidencia:143 [Mate]: hexagonal_spacer_MF_M3_H20_HEX5.5_FTD6_MTL6:3 ↔ ISO 4032 M3:13
- Coincidencia:144 [Mate]: ISO 4032 M3:16 ↔ base_nivel2:1
- Coincidencia:145 [Mate]: hexagonal_spacer_MF_M3_H20_HEX5.5_FTD6_MTL6:4 ↔ ISO 4032 M3:16
- Coincidencia:146 [Mate]: bateria:1 ↔ base_chasis_v4-dimsAjustadas:2
- Coincidencia:147 [Mate]: hexagonal_spacer_MF_M3_H10_HEX5.5_FTD6_MTL6:1 ↔ base_chasis_v4-dimsAjustadas:2
- Coincidencia:148 [Mate]: hexagonal_spacer_MF_M3_H10_HEX5.5_FTD6_MTL6:2 ↔ base_chasis_v4-dimsAjustadas:2
- Coincidencia:149 [Mate]: hexagonal_spacer_MF_M3_H10_HEX5.5_FTD6_MTL6:1 ↔ base_chasis_v4-dimsAjustadas:2
- Coincidencia:150 [Mate]: hexagonal_spacer_MF_M3_H10_HEX5.5_FTD6_MTL6:2 ↔ base_chasis_v4-dimsAjustadas:2
- Coincidencia:151 [Mate]: ISO 4762 M3 x 8:10 ↔ base_chasis_v4-dimsAjustadas:2
- Coincidencia:152 [Mate]: ISO 4762 M3 x 8:10 ↔ base_chasis_v4-dimsAjustadas:2
- Coincidencia:153 [Mate]: ISO 4762 M3 x 8:9 ↔ base_chasis_v4-dimsAjustadas:2
- Coincidencia:154 [Mate]: ISO 4762 M3 x 8:9 ↔ base_chasis_v4-dimsAjustadas:2
- Coincidencia:161 [Mate]: motor:1 ↔ base_chasis_v4-dimsAjustadas:2
- Coincidencia:163 [Mate]: motor:1 ↔ llanta:1
- Coincidencia:164 [Mate]: motor:1 ↔ llanta:1
- Coincidencia:169 [Mate]: motor:2 ↔ base_chasis_v4-dimsAjustadas:2
- Coincidencia:171 [Mate]: motor:2 ↔ llanta:2
- Coincidencia:172 [Mate]: motor:2 ↔ llanta:2
- Coincidencia:174 [Mate]: ISO 4762 M3 x 8:14 ↔ ideaboard:1
- Coincidencia:175 [Mate]: hexagonal_spacer_MF_M3_H06_HEX5.5_FTD3_MTL6:8 ↔ ISO 4762 M3 x 8:14
- Coincidencia:176 [Mate]: ISO 4762 M3 x 8:11 ↔ ideaboard:1
- Coincidencia:177 [Mate]: hexagonal_spacer_MF_M3_H06_HEX5.5_FTD3_MTL6:7 ↔ ISO 4762 M3 x 8:11
- Coincidencia:178 [Mate]: ISO 4762 M3 x 8:13 ↔ ideaboard:1
- Coincidencia:179 [Mate]: hexagonal_spacer_MF_M3_H06_HEX5.5_FTD3_MTL6:6 ↔ ISO 4762 M3 x 8:13
- Coincidencia:180 [Mate]: ISO 4762 M3 x 8:12 ↔ ideaboard:1
- Coincidencia:181 [Mate]: hexagonal_spacer_MF_M3_H06_HEX5.5_FTD3_MTL6:5 ↔ ISO 4762 M3 x 8:12
- Coincidencia:183 [Mate]: ISO 4762 M2 x 8:10 ↔ base_chasis_v4-dimsAjustadas:2
- Coincidencia:185 [Mate]: ISO 4762 M2 x 8:7 ↔ base_chasis_v4-dimsAjustadas:2
- Coincidencia:187 [Mate]: ISO 4762 M2 x 8:9 ↔ base_chasis_v4-dimsAjustadas:2
- Coincidencia:189 [Mate]: ISO 4762 M2 x 8:8 ↔ base_chasis_v4-dimsAjustadas:2
- Coincidencia:190 [Mate]: ISO 4032 M2:12 ↔ base_chasis_v4-dimsAjustadas:2
- Coincidencia:191 [Mate]: ISO 4032 M2:12 ↔ ISO 4762 M2 x 8:8
- Coincidencia:192 [Mate]: ISO 4032 M2:13 ↔ base_chasis_v4-dimsAjustadas:2
- Coincidencia:193 [Mate]: ISO 4032 M2:13 ↔ ISO 4762 M2 x 8:9
- Coincidencia:194 [Mate]: ISO 4032 M2:15 ↔ base_chasis_v4-dimsAjustadas:2
- Coincidencia:195 [Mate]: ISO 4032 M2:15 ↔ ISO 4762 M2 x 8:7
- Coincidencia:196 [Mate]: ISO 4032 M2:14 ↔ base_chasis_v4-dimsAjustadas:2
- Coincidencia:197 [Mate]: ISO 4032 M2:14 ↔ ISO 4762 M2 x 8:10
- Coincidencia:205 [Mate]: Tower Pro MG90S Micro servo:2 ↔ Unidirectional shoulder:1
- Coincidencia:206 [Mate] (1 mm): Tower Pro MG90S Micro servo:2 ↔ Unidirectional shoulder:1
- Coincidencia:207 [Mate]: Tower Pro MG90S Micro servo:2 ↔ base_chasis_v4-dimsAjustadas:2
- Ángulo:1 [Angle] (0 deg): Tower Pro MG90S Micro servo:2 ↔ base_chasis_v4-dimsAjustadas:2
- Coincidencia:209 [Mate]: base_chasis_v4-dimsAjustadas:2
- Nivelación:211 [Flush]: base_chasis_v4-dimsAjustadas:2
- Coincidencia:210 [Mate]: base_chasis_v4-dimsAjustadas:2
- Ángulo:2 [Angle] (0 deg): bateria:1 ↔ base_chasis_v4-dimsAjustadas:2
- Ángulo:3 [Angle] (180 deg): switch:1 ↔ base_chasis_v4-dimsAjustadas:2
- Ángulo:4 [Angle] (180 deg): base_nivel2:1 ↔ sensorFrontal:2
- Ángulo:5 [Angle] (180 deg): base_nivel2:1 ↔ sensorFrontal:1
- Coincidencia:217 [Mate]: Tower Pro MG90S Micro servo:2 ↔ SujecionServo:1
- Coincidencia:226 [Mate]: SoporteMotor_3.0:2 ↔ base_chasis_v4-dimsAjustadas:2
- Coincidencia:227 [Mate]: motor:1 ↔ SoporteMotor_3.0:2
- Coincidencia:228 [Mate]: SoporteMotor_3.0:2 ↔ base_chasis_v4-dimsAjustadas:2
- Coincidencia:229 [Mate]: SoporteMotor_3.0:1 ↔ base_chasis_v4-dimsAjustadas:2
- Coincidencia:230 [Mate]: motor:2 ↔ SoporteMotor_3.0:1
- Coincidencia:231 [Mate]: SoporteMotor_3.0:1 ↔ base_chasis_v4-dimsAjustadas:2
- Tangente:5: motor:1 ↔ SoporteMotor_3.0:2
- Coincidencia:232 [Mate]: SoporteMotor_3.0:2 ↔ base_chasis_v4-dimsAjustadas:2
- Coincidencia:233 [Mate]: SoporteMotor_3.0:1 ↔ base_chasis_v4-dimsAjustadas:2
- Tangente:6: motor:2 ↔ SoporteMotor_3.0:1
- Insert:10: SS ISO 4762 M2,5 x 25:4 ↔ base_chasis_v4-dimsAjustadas:2
- Insert:12: SS ISO 4762 M2,5 x 25:6 ↔ base_chasis_v4-dimsAjustadas:2
- Insert:14: SS ISO 4762 M2,5 x 25:8 ↔ base_chasis_v4-dimsAjustadas:2
- Insert:15: SS ISO 4762 M2,5 x 25:9 ↔ base_chasis_v4-dimsAjustadas:2
- Insert:17: SS ISO 4762 M2,5 x 25:11 ↔ base_chasis_v4-dimsAjustadas:2
- Insert:18: SS ISO 4762 M2,5 x 25:12 ↔ base_chasis_v4-dimsAjustadas:2
- Nivelación:212 [Flush]: base_chasis_v4-dimsAjustadas:3 ↔ base_chasis_v4-dimsAjustadas:2
- Coincidencia:237 [Mate]: base_chasis_v4-dimsAjustadas:3 ↔ base_chasis_v4-dimsAjustadas:2
- Coincidencia:238 [Mate]: base_chasis_v4-dimsAjustadas:3 ↔ base_chasis_v4-dimsAjustadas:2
- Coincidencia:239 [Mate]: base_chasis_v4-dimsAjustadas:1 ↔ base_chasis_v4-dimsAjustadas:2
- Coincidencia:240 [Mate]: base_chasis_v4-dimsAjustadas:1 ↔ base_chasis_v4-dimsAjustadas:2
- Coincidencia:244 [Mate]: base_chasis_v4-dimsAjustadas:1 ↔ base_chasis_v4-dimsAjustadas:2
- Coincidencia:245 [Mate]: base_chasis_v4-dimsAjustadas:2 ↔ Bumper Delantero:1
- Coincidencia:246 [Mate]: base_chasis_v4-dimsAjustadas:2 ↔ Bumper Delantero:1
- Coincidencia:247 [Mate]: base_chasis_v4-dimsAjustadas:2 ↔ Bumper Delantero:1
- Coincidencia:248 [Mate]: Bumper Delantero:1 ↔ Esquineros Delanteros:1
- Coincidencia:249 [Mate]: base_chasis_v4-dimsAjustadas:2 ↔ Esquineros Delanteros:1
- Coincidencia:250 [Mate]: ISO 4762 M3 x 8:8 ↔ base_nivel2:1
- Coincidencia:251 [Mate]: ISO 4762 M3 x 8:8 ↔ base_nivel2:1
- Coincidencia:252 [Mate]: Bumper Delantero:1 ↔ Esquineros Delanteros:1
- Coincidencia:253 [Mate]: PARED TRASERA:1 ↔ base_chasis_v4-dimsAjustadas:2
- Coincidencia:254 [Mate]: PARED TRASERA:1 ↔ base_chasis_v4-dimsAjustadas:1
- Coincidencia:255 [Mate]: PAREDES LATERALES:2 ↔ base_chasis_v4-dimsAjustadas:2
- Coincidencia:256 [Mate]: PAREDES LATERALES:2 ↔ base_chasis_v4-dimsAjustadas:3
- Coincidencia:257 [Mate]: PAREDES LATERALES:2 ↔ Esquineros Delanteros:1
- Coincidencia:258 [Mate]: PARED FRONTAL:1 ↔ base_chasis_v4-dimsAjustadas:2
- Coincidencia:259 [Mate]: PARED FRONTAL:1 ↔ Bumper Delantero:1
- Coincidencia:260 [Mate]: PARED FRONTAL:1 ↔ Esquineros Delanteros:1
- Coincidencia:261 [Mate]: base_chasis_v4-dimsAjustadas:3 ↔ Techo Armadura:1
- Coincidencia:262 [Mate]: base_chasis_v4-dimsAjustadas:2 ↔ Techo Armadura:1
- Coincidencia:263 [Mate]: base_chasis_v4-dimsAjustadas:3 ↔ Techo Armadura:1
- Coincidencia:264 [Mate]: base_chasis_v4-dimsAjustadas:3 ↔ Techo Armadura:1
- Nivelación:213 [Flush]: Pieza de Silicona:1 ↔ Techo Armadura:1
- Coincidencia:268 [Mate]: Pieza de Silicona:1 ↔ Techo Armadura:1
- Coincidencia:269 [Mate]: PARED FRONTAL:1 ↔ Esquineros Delanteros:1
- Coincidencia:270 [Mate]: base_chasis_v4-dimsAjustadas:2 ↔ Guardabarros:1
- Coincidencia:272 [Mate]: llanta:1 ↔ Guardabarros:1
- Coincidencia:273 [Mate]: base_chasis_v4-dimsAjustadas:2 ↔ Guardabarros:1
- Coincidencia:274 [Mate]: ISO 4762 M3 x 8:12 ↔ base_nivel2:1
- Coincidencia:275 [Mate]: hexagonal_spacer_MF_M3_H06_HEX5.5_FTD3_MTL6:6 ↔ base_nivel2:1
- Coincidencia:276 [Mate]: hexagonal_spacer_MF_M3_H06_HEX5.5_FTD3_MTL6:6 ↔ base_nivel2:1
- Coincidencia:277 [Mate]: hexagonal_spacer_MF_M3_H06_HEX5.5_FTD3_MTL6:6 ↔ base_nivel2:1
- Coincidencia:278 [Mate]: hexagonal_spacer_MF_M3_H06_HEX5.5_FTD3_MTL6:6 ↔ base_nivel2:1
- Coincidencia:279 [Mate]: hexagonal_spacer_MF_M3_H06_HEX5.5_FTD3_MTL6:6 ↔ base_nivel2:1
- Coincidencia:280 [Mate]: hexagonal_spacer_MF_M3_H06_HEX5.5_FTD3_MTL6:6 ↔ base_nivel2:1
- Coincidencia:281 [Mate]: hexagonal_spacer_MF_M3_H06_HEX5.5_FTD3_MTL6:6 ↔ base_nivel2:1
- Coincidencia:282 [Mate]: SS ISO 4762 M2,5 x 25:12 ↔ sensorInferior:3
- Coincidencia:283 [Mate]: ISO 4762 M3 x 12:1 ↔ sensorInferior:3
- Coincidencia:284 [Mate]: sensorInferior:3 ↔ base_chasis_v4-dimsAjustadas:2
- Coincidencia:285 [Mate]: ISO 4762 M3 x 8:9 ↔ base_chasis_v4-dimsAjustadas:2
- Coincidencia:286 [Mate]: base_chasis_v4-dimsAjustadas:2 ↔ PresaPilotInventorVersion:1
- Coincidencia:287 [Mate]: base_chasis_v4-dimsAjustadas:2 ↔ PresaPilotInventorVersion:1
- Coincidencia:288 [Mate]: PresaPilotInventorVersion:1
- Coincidencia:289 [Mate]: hexagonal_spacer_MF_M3_H20_HEX5.5_FTD6_MTL6:5 ↔ base_chasis_v4-dimsAjustadas:2
- Coincidencia:290 [Mate]: hexagonal_spacer_MF_M3_H20_HEX5.5_FTD6_MTL6:5 ↔ base_chasis_v4-dimsAjustadas:2
- Nivelación:215 [Flush]: BaseMotorSetJose:1
- Coincidencia:291 [Mate]: Acrilicos Superiores:1 ↔ Esquineros Delanteros:1
- Coincidencia:292 [Mate]: Acrilicos Superiores:1 ↔ Techo Armadura:1
- Nivelación:216 [Flush] (6 mm): Acrilicos Superiores:1
- Nivelación:219 [Flush]: DistanciaSpacer3mm:1 ↔ PARED FRONTAL:1
- Coincidencia:293 [Mate]: EnsambleGarraSTD:1 ↔ DistanciaSpacer3mm:1
- Nivelación:220 [Flush]: EnsambleGarraSTD:1 ↔ Bumper Delantero:1
- Coincidencia:294 [Mate]: EnsambleGarraSTD:1
- Nivelación:222 [Flush]: EnsambleGarraSTD:1 ↔ EjeMotor:1
- Coincidencia:295 [Mate]: Acrilicos Superiores:1 ↔ Techo Armadura:1
- Coincidencia:296 [Mate]: Acrilicos Superiores:1 ↔ Techo Armadura:1
- Coincidencia:297 [Mate]: Acrilicos Superiores:1 ↔ Techo Armadura:1
- Coincidencia:298 [Mate]: Acrilicos Superiores:1 ↔ Techo Armadura:1
- Ángulo:6 [Angle] (0 deg): Techo Armadura:1
- Ángulo:7 [Angle] (180 deg): EnsambleBaseMotor_Mediciones
- Coincidencia:299 [Mate] (6 mm): EnsambleBaseMotor_Mediciones ↔ Acrilicos Superiores:1
- Coincidencia:300 [Mate]: EnsambleBaseMotor_Mediciones ↔ base_chasis_v4-dimsAjustadas:2
- Ángulo:8 [Angle] (180 deg): EnsambleBaseMotor_Mediciones
